# Autodesk Inventor assembly: CollectorHolderAssembly
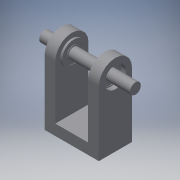
[picture p0: Inventor's stored thumbnail of the model, 180x180]
Saved by Autodesk Inventor 2017 (Build 210142000, 142)
## iProperties
Created: 2017-04-19
Part Number: CollectorHolderAssembly
Document SubType Name: Assembly
Designer: User
Author: User
## Documents named in this file (4)
- C:\Robotics\CAD\2016-17_CAD\CollectorHolderAssembly.iam
- C:\Robotics\CAD\2016-17_CAD\CollectorHolder.ipt
- C:\Robotics\CAD\2016-17_CAD\Axle2.11.ipt
- C:\Robotics\CAD\COTSParts\Actobotics\535 parts\535198.ipt
## Components (4 placed, 3 different names)
1. CollectorHolder:1 — Insert:1, Insert:2, Insert:3
2. Axle2.11:1 — Insert:3
3. 535198:1 — Insert:1
4. 535198:2 — Insert:2
## Relationships (3: Insert 3)
- Insert:1: CollectorHolder:1 ↔ 535198:1
- Insert:2: CollectorHolder:1 ↔ 535198:2
- Insert:3 (-9.779 mm): CollectorHolder:1 ↔ Axle2.11:1
